# Autodesk Inventor assembly: SestavaKamera
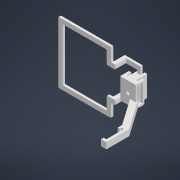
[picture p0: Inventor's stored thumbnail of the model, 180x180]
Saved by Autodesk Inventor 2022 (Build 260153000, 153)
## iProperties
Created: 2023-04-13
Part Number: SestavaKamera
Document SubType Name: Assembly
Designer: tada
Author: tada
## Documents named in this file (3)
- C:\Users\tadea\Documents\3D-tisk\Maturita\SestavaKamera.iam
- C:\Users\tadea\Documents\3D-tisk\Maturita\DrzakLEDky.ipt
- C:\Users\tadea\Documents\3D-tisk\Maturita\DrzakKamera.ipt
## Components (2 placed, 2 different names)
1. DrzakLEDky:1 — Proti sobě:1, Proti sobě:2
2. DrzakKamera:1 — Proti sobě:1, Proti sobě:2
## Relationships (2: Mate 2)
- Proti sobě:1 [Mate]: DrzakLEDky:1 ↔ DrzakKamera:1
- Proti sobě:2 [Mate]: DrzakLEDky:1 ↔ DrzakKamera:1
